# Autodesk Inventor assembly: 20mm T-Nut Fastener 1764
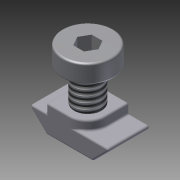
[picture p0: Inventor's stored thumbnail of the model, 180x180]
Saved by Autodesk Inventor 2011 (Build 150239000, 239)
## iProperties
Created: 2011-02-18
Part Number: 20mm T-Nut Fastener 1764
Document SubType Name: Assembly
Designer: dfranz
Author: dfranz
## Documents named in this file (3)
- R:\CAD Archives\Frame Systems\Aluminum Extrusion 1764\T-Nuts 1764\20mm T-Nut Fastener 1764.iam
- R:\CAD Archives\Frame Systems\Aluminum Extrusion 1764\T-Nuts 1764\20mm T-Nut 1764.ipt
- R:\CAD Archives\Frame Systems\Aluminum Extrusion 1764\T-Nuts 1764\20mm T-Nut Fastener 1764.ipt
## Components (2 placed, 2 different names)
1. 20mm T-Nut 1764:1 — Insert:1
2. 20mm T-Nut Fastener 1764:1 — Insert:1
## Relationships (1: Insert 1)
- Insert:1 (4.5466 mm): 20mm T-Nut 1764:1 ↔ 20mm T-Nut Fastener 1764:1
